# Autodesk Inventor assembly: axc40sg12__-r9-300-461-__-__-00-_-_-l1l
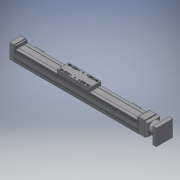
[picture p0: Inventor's stored thumbnail of the model, 180x180]
Saved by Autodesk Inventor 2018 (Build 220112000, 112)
## iProperties
Company: TraceParts S.A.
Created: 2020-05-30
Part Number: axc40sg12__-r9-300-461-__-__-00-_-_-l1l
Checked By: TraceParts S.A.
Catalog Web Link: www.traceparts.com
Document SubType Name: Assembly
Designer: TraceParts
REFERENCE: AXC40SG12__-R9-300-461-__-__-00-_-_
DESIGN: 02 - asse lineare con transmissione a vite e guida a ricircolo di sfere AXC40-S
SUPPLIER: NADELLA
TraceParts.PartNumber: 32-15042009-081775
TraceParts.PartTitle: 02 - asse lineare con transmissione a vite e guida a ricircolo di sfere AXC40-S
TraceParts.InstanceId: 32-15042009-0817752JS3SDS5NK9W6X5NKLHCUIRSQ
TraceParts.PartStatus: Published
TraceParts.PartVersion: 1.1.4
TRACEPARTS: TRACEPARTS
TraceParts.PartLanguage: it
TraceParts.ClassPath: NADELLA:32-15042009-081775
Author: TraceParts
## Documents named in this file (5)
- C:\Users\Francesco\no-brim\Meccanica\Progetto Inventor no-brim\Parti\Asse lineare corsa 300 mm\Assieme asse lineare corsa 300 mm.iam
- C:\Users\Francesco\no-brim\Meccanica\Progetto Inventor no-brim\Parti\Asse lineare corsa 300 mm\axc40sg12__-r9-300-461-__-__-00-_-_-l1l_01.ipt
- C:\Users\Francesco\no-brim\Meccanica\Progetto Inventor no-brim\Parti\Asse lineare corsa 300 mm\axc40sg12__-r9-300-461-__-__-00-_-_-l1l_02.ipt
- C:\Users\Francesco\no-brim\Meccanica\Progetto Inventor no-brim\Parti\Asse lineare corsa 300 mm\axc40sg12__-r9-300-461-__-__-00-_-_-l1l_03.ipt
- C:\Users\Francesco\no-brim\Meccanica\Progetto Inventor no-brim\Parti\Asse lineare corsa 300 mm\axc40sg12__-r9-300-461-__-__-00-_-_-l1l_04.ipt
## Components (4 placed, 4 different names)
1. axc40sg12__-r9-300-461-__-__-00-_-_-l1l_01:1 — Allineato:1, Coincidente:1, Coincidente:2
2. axc40sg12__-r9-300-461-__-__-00-_-_-l1l_02:1 — Allineato:1, Coincidente:1, Coincidente:2
3. axc40sg12__-r9-300-461-__-__-00-_-_-l1l_03:1
4. axc40sg12__-r9-300-461-__-__-00-_-_-l1l_04:1
## Relationships (3: Mate 2, Flush 1)
- Allineato:1 [Flush] (0.5 mm): axc40sg12__-r9-300-461-__-__-00-_-_-l1l_01:1 ↔ axc40sg12__-r9-300-461-__-__-00-_-_-l1l_02:1
- Coincidente:1 [Mate]: axc40sg12__-r9-300-461-__-__-00-_-_-l1l_01:1 ↔ axc40sg12__-r9-300-461-__-__-00-_-_-l1l_02:1
- Coincidente:2 [Mate]: axc40sg12__-r9-300-461-__-__-00-_-_-l1l_01:1 ↔ axc40sg12__-r9-300-461-__-__-00-_-_-l1l_02:1
